# Autodesk Inventor assembly: NUCLEO-F411RE-full
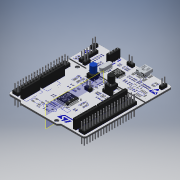
[picture p0: Inventor's stored thumbnail of the model, 180x180]
Saved by Autodesk Inventor 2017.3 (Build 213256000, 256)
## iProperties
Created: 2015-02-26
Part Number: NUCLEO-F411RE-full
Material: Generisch
Description: STEP AP214
Document SubType Name: Assembly
Designer: Nils
Sending System: o
Preprocessor: o
Title: NUCLEO-F411RE.STEP
Revision Number: ANY
## Documents named in this file (24)
- C:\Users\Nils\Documents\GitHub\Eurobot2018\Hardware\Roboterplatform\Nucleo-simplified\NUCLEO-F411RE-simplified.iam
- C:\Users\Nils\Documents\GitHub\Eurobot2018\Hardware\Roboterplatform\Nucleo-simplified\NUCLEO-F411RE_PCB_Varsaylan.ipt
- C:\Users\Nils\Documents\GitHub\Eurobot2018\Hardware\Roboterplatform\Nucleo-simplified\NUCLEO-F411RE_PCB_TOP_Solder_Varsaylan.ipt
- C:\Users\Nils\Documents\GitHub\Eurobot2018\Hardware\Roboterplatform\Nucleo-simplified\NUCLEO-F411RE_PCB_BOTTOM_Solder_Varsaylan.ipt
- C:\Users\Nils\Documents\GitHub\Eurobot2018\Hardware\Roboterplatform\Nucleo-simplified\NUCLEO-F411RE_PCB_TOP_Overlay_Varsaylan.ipt
- C:\Users\Nils\Documents\GitHub\Eurobot2018\Hardware\Roboterplatform\Nucleo-simplified\NUCLEO-F411RE_PCB_TOP_Designators_Varsaylan.ipt
- C:\Users\Nils\Documents\GitHub\Eurobot2018\Hardware\Roboterplatform\Nucleo-simplified\NUCLEO-F411RE_PCB_BOTTOM_Overlay_Varsaylan.ipt
- C:\Users\Nils\Documents\GitHub\Eurobot2018\Hardware\Roboterplatform\Nucleo-simplified\SAMTEC_SSQ-106-01-G-S_for_NUCLEO_Varsaylan.ipt
- C:\Users\Nils\Documents\GitHub\Eurobot2018\Hardware\Roboterplatform\Nucleo-simplified\SAMTEC_SSQ-108-01-G-S_for_NUCLEO_Varsaylan.ipt
- C:\Users\Nils\Documents\GitHub\Eurobot2018\Hardware\Roboterplatform\Nucleo-simplified\SAMTEC_SSQ-110-01-G-S_for_NUCLEO_Varsaylan.ipt
- C:\Users\Nils\Documents\GitHub\Eurobot2018\Hardware\Roboterplatform\Nucleo-simplified\MOLEX_0678038020_for_NUCLEO.ipt
- C:\Users\Nils\Documents\GitHub\Eurobot2018\Hardware\Roboterplatform\Nucleo-simplified\SAMTEC_TSW-119-07-T-D_for_NUCLEO_Varsaylan.ipt
- C:\Users\Nils\Documents\GitHub\Eurobot2018\Hardware\Roboterplatform\Nucleo-simplified\SAMTEC_TSW-102-07-T-S_for_NUCLEO_Varsaylan.ipt
- C:\Users\Nils\Documents\GitHub\Eurobot2018\Hardware\Roboterplatform\Nucleo-simplified\SAMTEC_TSW-103-07-T-S_for_NUCLEO_Varsaylan.ipt
- C:\Users\Nils\Documents\GitHub\Eurobot2018\Hardware\Roboterplatform\Nucleo-simplified\SAMTEC_TSW-104-07-T-S_for_NUCLEO_Varsaylan.ipt
- C:\Users\Nils\Documents\GitHub\Eurobot2018\Hardware\Roboterplatform\Nucleo-simplified\SAMTEC_TSW-106-07-T-S_for_NUCLEO_Varsaylan.ipt
- C:\Users\Nils\Documents\GitHub\Eurobot2018\Hardware\Roboterplatform\Nucleo-simplified\MOLEX_90059-0007.ipt
- C:\Users\Nils\Documents\GitHub\Eurobot2018\Hardware\Roboterplatform\Nucleo-simplified\ST_STM32F411RET6_Varsaylan.ipt
- C:\Users\Nils\Documents\GitHub\Eurobot2018\Hardware\Roboterplatform\Nucleo-simplified\ST_STM32F103CBT6_Varsaylan.ipt
- C:\Users\Nils\Documents\GitHub\Eurobot2018\Hardware\Roboterplatform\Nucleo-simplified\ESWITCH_TL3301SPF160QGBLK_Varsaylan.ipt
- C:\Users\Nils\Documents\GitHub\Eurobot2018\Hardware\Roboterplatform\Nucleo-simplified\ESWITCH_TL3301SPF160QGBLU_Varsaylan.ipt
- C:\Users\Nils\Documents\GitHub\Eurobot2018\Hardware\Roboterplatform\Nucleo-simplified\ST_STS7PF30L_Varsaylan.ipt
- C:\Users\Nils\Documents\GitHub\Eurobot2018\Hardware\Roboterplatform\Nucleo-simplified\ABRACON_ABL-8.000MHZ-B2_Varsaylan.ipt
- C:\Users\Nils\Documents\GitHub\Eurobot2018\Hardware\Roboterplatform\Nucleo-simplified\ST_LD1117S50TR_Varsaylan.ipt
## Components (31 placed, 31 different names)
1. NAUO1
2. NAUO4
3. NAUO6
4. NAUO7
5. NAUO8
6. NAUO9
7. NAUO10
8. NAUO11
9. NAUO12
10. NAUO13
11. NAUO14
12. NAUO15 — Symmetrie:1
13. NAUO16 — Symmetrie:1
14. NAUO17
15. NAUO18
16. NAUO19
17. NAUO20
18. NAUO21
19. NAUO22
20. NAUO23
21. NAUO24
22. NAUO25
23. NAUO26
24. NAUO27
25. NAUO28
26. NAUO29
27. NAUO30
28. NAUO31
29. NAUO32
30. NAUO33
31. NAUO41
## Relationships (1: Symmetry 1)
- Symmetrie:1: NAUO15 ↔ NAUO16
